# Autodesk Inventor assembly: Roller_Bracket
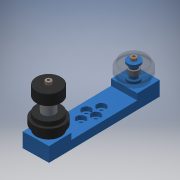
[picture p0: Inventor's stored thumbnail of the model, 180x180]
Saved by Autodesk Inventor 2019.4 (Build 234330000, 330)
## iProperties
Created: 2021-02-01
Part Number: Roller_Bracket
Document SubType Name: Assembly
Designer: Jorian Brusind
Mass: 44.0669 g
Surface Area: 169.812 cm^2
Volume: 42.4218 cm^3
Density: 1.03878 g/cm^3
Author: Jorian Brusind
## Documents named in this file (9)
- C:\Users\Jorian Brusind\Documents\GitHub\PersonalProjects\HyperRail\Inventor Files\Roller_Bracket.iam
- C:\Users\Jorian Brusind\Documents\GitHub\PersonalProjects\HyperRail\Inventor Files\RollerWheel.ipt
- C:\Users\Jorian Brusind\Documents\GitHub\PersonalProjects\Inventor Projects\Useful models\Metric bolt\Bolt M3 25mm.ipt
- C:\Users\Jorian Brusind\Documents\GitHub\PersonalProjects\Inventor Projects\Useful models\683ZZBallBearing.ipt
- C:\Users\Jorian Brusind\Documents\GitHub\PersonalProjects\HyperRail\Inventor Files\Back_Bracket.ipt
- C:\Users\Jorian Brusind\Documents\GitHub\PersonalProjects\HyperRail\Inventor Files\3mmSpacer.ipt
- C:\Users\Jorian Brusind\Documents\GitHub\PersonalProjects\HyperRail\Inventor Files\Idlepulley_Spacer.ipt
- C:\Users\Jorian Brusind\Documents\GitHub\PersonalProjects\HyperRail\Inventor Files\11mm_BearingWheel.ipt
- C:\Users\Jorian Brusind\Documents\GitHub\PersonalProjects\Inventor Projects\Useful models\Metric bolt\Bolt M3 50mm.ipt
## Components (13 placed, 8 different names)
1. RollerWheel:1 — Mate:3, Flush:3
2. RollerWheel:2 — Mate:6, Flush:2, Mate:17
3. Bolt M3 25mm:1 — Mate:4, Mate:20, Mate:21, Mate:24, Mate:25
4. 683ZZBallBearing:1 — Mate:3, Mate:4, Flush:3, Mate:22, Mate:23
5. 683ZZBallBearing:2 — Mate:6, Flush:2, Mate:18, Mate:19
6. 3mmSpacer:1 — Mate:18, Mate:29, Mate:30
7. 3mmSpacer:2 — Mate:17, Mate:19, Mate:28
8. 3mmSpacer:3 — Mate:20, Mate:22, Mate:24
9. 3mmSpacer:4 — Mate:21, Mate:23, Mate:27
10. Back_Bracket:1 — Mate:25, Mate:27, Mate:28
11. Idlepulley_Spacer:1 — Mate:29, Mate:30, Mate:32, Mate:33
12. 11mm_BearingWheel:1 — Mate:32, Mate:34
13. Bolt M3 50mm:1 — Mate:33, Mate:34
## Relationships (21: Mate 19, Flush 2)
- Mate:3: RollerWheel:1 ↔ 683ZZBallBearing:1
- Mate:4: Bolt M3 25mm:1 ↔ 683ZZBallBearing:1
- Mate:6: RollerWheel:2 ↔ 683ZZBallBearing:2
- Flush:2 (5.5 mm): RollerWheel:2 ↔ 683ZZBallBearing:2
- Mate:17: RollerWheel:2 ↔ 3mmSpacer:2
- Mate:18: 683ZZBallBearing:2 ↔ 3mmSpacer:1
- Mate:19: 683ZZBallBearing:2 ↔ 3mmSpacer:2
- Flush:3 (5.5 mm): RollerWheel:1 ↔ 683ZZBallBearing:1
- Mate:20: Bolt M3 25mm:1 ↔ 3mmSpacer:3
- Mate:21: Bolt M3 25mm:1 ↔ 3mmSpacer:4
- Mate:22: 683ZZBallBearing:1 ↔ 3mmSpacer:3
- Mate:23: 683ZZBallBearing:1 ↔ 3mmSpacer:4
- Mate:24: Bolt M3 25mm:1 ↔ 3mmSpacer:3
- Mate:25: Bolt M3 25mm:1 ↔ Back_Bracket:1
- Mate:27 (1 mm): 3mmSpacer:4 ↔ Back_Bracket:1
- Mate:28 (1 mm): 3mmSpacer:2 ↔ Back_Bracket:1
- Mate:29: 3mmSpacer:1 ↔ Idlepulley_Spacer:1
- Mate:30: 3mmSpacer:1 ↔ Idlepulley_Spacer:1
- Mate:32: Idlepulley_Spacer:1 ↔ 11mm_BearingWheel:1
- Mate:33: Idlepulley_Spacer:1 ↔ Bolt M3 50mm:1
- Mate:34: 11mm_BearingWheel:1 ↔ Bolt M3 50mm:1
